# Autodesk Inventor assembly: Full_Assembly
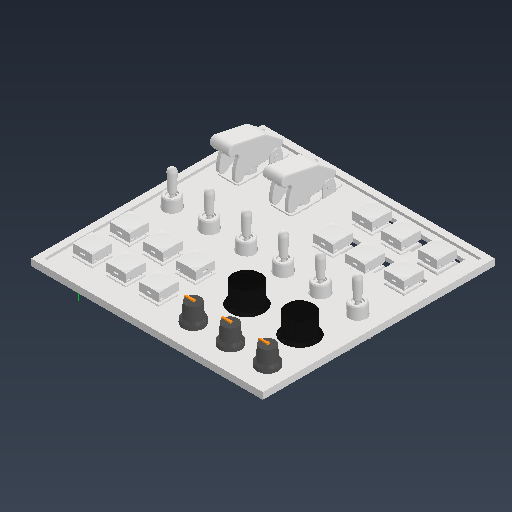
[picture p0: Inventor's stored thumbnail of the model, 512x512]
Saved by Autodesk Inventor 2025.3 (Build 293356000, 356)
## iProperties
Created: 2025-09-08
Part Number: Full_Assembly
Document SubType Name: Assembly
Designer: tolga
Author: tolga
## Documents named in this file (10)
- C:\Users\tolga\Documents\Repositories\Personal Projects\Sim-Control-Panel-v1.0\CAD\Full_Assembly.iam
- C:\Users\tolga\Documents\Repositories\Personal Projects\Sim-Control-Panel-v1.0\CAD\3rd_Party_Parts\Lighted_Buttons\Lighted_Buttons.iam
- C:\Users\tolga\Documents\Repositories\Personal Projects\Sim-Control-Panel-v1.0\CAD\3rd_Party_Parts\On-On Switch.ipt
- C:\Users\tolga\Documents\Repositories\Personal Projects\Sim-Control-Panel-v1.0\CAD\3rd_Party_Parts\Momentary Switch.ipt
- C:\Users\tolga\Documents\Repositories\Personal Projects\Sim-Control-Panel-v1.0\CAD\3rd_Party_Parts\Encoder_Knob.ipt
- C:\Users\tolga\Documents\Repositories\Personal Projects\Sim-Control-Panel-v1.0\CAD\3rd_Party_Parts\Potentiometer Knob.ipt
- C:\Users\tolga\Documents\Repositories\Personal Projects\Sim-Control-Panel-v1.0\CAD\3rd_Party_Parts\Switch Guard.ipt
- C:\Users\tolga\Documents\Repositories\Personal Projects\Sim-Control-Panel-v1.0\CAD\Faceplate.ipt
- C:\Users\tolga\Documents\Repositories\Personal Projects\Sim-Control-Panel-v1.0\CAD\3rd_Party_Parts\PEC12R-4125F-N0012.ipt
- C:\Users\tolga\Documents\Repositories\Personal Projects\Sim-Control-Panel-v1.0\CAD\3rd_Party_Parts\PDB12-H4201-103BF\PDB12-H4201-103BF.iam
## Components (33 placed, 9 different names)
1. Lighted_Buttons:1 [sub-assembly] — Mate:1, Mate:2
2. Lighted_Buttons:2 [sub-assembly]
3. Lighted_Buttons:3 [sub-assembly]
4. Lighted_Buttons:4 [sub-assembly]
5. Lighted_Buttons:5 [sub-assembly] — Mate:3, Mate:4
6. Lighted_Buttons:6 [sub-assembly]
7. Lighted_Buttons:7 [sub-assembly] — Mate:7, Mate:8
8. Lighted_Buttons:8 [sub-assembly] — Mate:9, Mate:10
9. Lighted_Buttons:9 [sub-assembly]
10. Lighted_Buttons:10 [sub-assembly]
11. Lighted_Buttons:11 [sub-assembly] — Mate:11, Mate:12
12. Lighted_Buttons:12 [sub-assembly] — Mate:5, Mate:6
13. On-On Switch:1 — Insert:1, Insert:20
14. Momentary Switch:1 — Insert:14
15. Momentary Switch:2 — Insert:15
16. Momentary Switch:3 — Insert:16
17. Encoder_Knob:1 — Insert:3, Insert:4
18. Momentary Switch:4 — Insert:19
19. Momentary Switch:5 — Insert:17
20. Momentary Switch:6 — Insert:18
21. Switch Guard:1 — Insert:1
22. On-On Switch:2 — Insert:21
23. Switch Guard:3
24. Faceplate:1 — Insert:4, Insert:9, Insert:10, Insert:11, Insert:13, Insert:14, Insert:15, Insert:16, Insert:17, Insert:18, Insert:19, Insert:20, Insert:21, Mate:1, Mate:2, Mate:3, Mate:4, Mate:5, Mate:6, Mate:7, Mate:8, Mate:9, Mate:10, Mate:11, Mate:12
25. PEC12R-4125F-N0012:1 — Insert:3
26. PDB12-H4201-103BF:3 [sub-assembly] — Insert:6
27. Potentiometer Knob:4 — Insert:6, Insert:9
28. PDB12-H4201-103BF:4 [sub-assembly]
29. Potentiometer Knob:5 — Insert:10
30. PDB12-H4201-103BF:5 [sub-assembly]
31. Potentiometer Knob:6 — Insert:11
32. Encoder_Knob:2 — Insert:13
33. PEC12R-4125F-N0012:2
## Relationships (32: Insert 20, Mate 12)
- Insert:1 (5 mm): On-On Switch:1 ↔ Switch Guard:1
- [Insert] (5 mm): On-On Switch:2 ↔ Switch Guard:3
- Insert:3 (1 mm): Encoder_Knob:1 ↔ PEC12R-4125F-N0012:1
- Insert:4: Encoder_Knob:1 ↔ Faceplate:1
- Insert:6: PDB12-H4201-103BF:3 ↔ Potentiometer Knob:4
- [Insert]: PDB12-H4201-103BF:4 ↔ Potentiometer Knob:5
- [Insert]: PDB12-H4201-103BF:5 ↔ Potentiometer Knob:6
- Insert:9: Faceplate:1 ↔ Potentiometer Knob:4
- Insert:10: Faceplate:1 ↔ Potentiometer Knob:5
- Insert:11: Faceplate:1 ↔ Potentiometer Knob:6
- [Insert] (1 mm): Encoder_Knob:2 ↔ PEC12R-4125F-N0012:2
- Insert:13: Faceplate:1 ↔ Encoder_Knob:2
- Insert:14: Momentary Switch:1 ↔ Faceplate:1
- Insert:15: Momentary Switch:2 ↔ Faceplate:1
- Insert:16: Momentary Switch:3 ↔ Faceplate:1
- Insert:17: Momentary Switch:5 ↔ Faceplate:1
- Insert:18: Momentary Switch:6 ↔ Faceplate:1
- Insert:19: Momentary Switch:4 ↔ Faceplate:1
- Insert:20: On-On Switch:1 ↔ Faceplate:1
- Insert:21: On-On Switch:2 ↔ Faceplate:1
- Mate:1: Lighted_Buttons:1 ↔ Faceplate:1
- Mate:2: Lighted_Buttons:1 ↔ Faceplate:1
- Mate:3: Lighted_Buttons:5 ↔ Faceplate:1
- Mate:4: Lighted_Buttons:5 ↔ Faceplate:1
- Mate:5: Lighted_Buttons:12 ↔ Faceplate:1
- Mate:6: Lighted_Buttons:12 ↔ Faceplate:1
- Mate:7: Lighted_Buttons:7 ↔ Faceplate:1
- Mate:8: Lighted_Buttons:7 ↔ Faceplate:1
- Mate:9: Lighted_Buttons:8 ↔ Faceplate:1
- Mate:10: Lighted_Buttons:8 ↔ Faceplate:1
- Mate:11: Lighted_Buttons:11 ↔ Faceplate:1
- Mate:12: Lighted_Buttons:11 ↔ Faceplate:1
## Named parameters: d1_d0 = 5 mm, d26_d25 = 0 mm, d27_d25 = 0 mm, d31_d22 = 1 mm
